# Autodesk Inventor assembly: Test_zebatek_odl_rowna_srednicy
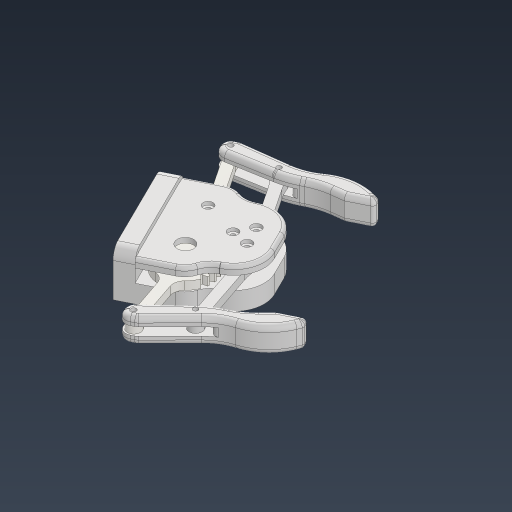
[picture p0: Inventor's stored thumbnail of the model, 512x512]
Saved by Autodesk Inventor 2024 (Build 280153000, 153)
## iProperties
Created: 2023-12-19
Part Number: Test_zebatek_odl_rowna_srednicy
Document SubType Name: Assembly
Designer: Piter
Author: Piter
## Documents named in this file (8)
- C:\Users\Piter\OneDrive\Pulpit\Modele\My-3D-printing-projects\gripper\Mygripper\Test_chwytaka.iam
- C:\Users\Piter\OneDrive\Pulpit\Modele\My-3D-printing-projects\gripper\Mygripper\Zebatka_servo.ipt
- C:\Users\Piter\OneDrive\Pulpit\Modele\My-3D-printing-projects\gripper\Mygripper\Podstawa.ipt
- C:\Users\Piter\OneDrive\Pulpit\Modele\My-3D-printing-projects\gripper\Mygripper\Connector.ipt
- C:\Users\Piter\OneDrive\Pulpit\Modele\My-3D-printing-projects\gripper\Mygripper\szczeka.ipt
- C:\Users\Piter\OneDrive\Pulpit\Modele\My-3D-printing-projects\gripper\Mygripper\Zebatka_bez_servo.ipt
- C:\Users\Piter\OneDrive\Pulpit\Modele\My-3D-printing-projects\gripper\Mygripper\Spacer.ipt
- C:\Users\Piter\OneDrive\Pulpit\Modele\My-3D-printing-projects\gripper\Mygripper\Top.ipt
## Components (9 placed, 6 different names)
1. Spur Gear2:2 — Rotational:1, Rotational:4, Mate:1, Mate:3, Rotational:5, Rotational:10, Rotation:1
2. Podstawa:1 — Rotational:1, Rotational:3, Rotational:4, Rotational:8, Rotational:9, Rotational:10, Rigid:1, Mate:7, Mate:8, Mate:9
3. Connector:1 — Rotational:3, Mate:2, Mate:4
4. Connector:2 — Rotational:8, Mate:5
5. szczeka:1 — Mate:1, Mate:2, Mate:3, Rotational:5, Mate:4
6. szczeka:2 — Mate:5, Mate:6
7. Spur Gear2:3 — Rotational:9, Mate:6, Rotation:1
8. Spacer:1 — Rigid:1
9. Top:1 — Mate:7, Mate:8, Mate:9
## Relationships (18: Mate 9, RevoluteJoint 7, RelateRotation 1, WeldJoint 1)
- Rotational:1 [RevoluteJoint]: Spur Gear2:2 ↔ Podstawa:1
- Rotational:3 [RevoluteJoint]: Podstawa:1 ↔ Connector:1
- Rotational:4 [RevoluteJoint]: Spur Gear2:2 ↔ Podstawa:1
- Mate:1: Spur Gear2:2 ↔ szczeka:1
- Mate:2: Connector:1 ↔ szczeka:1
- Mate:3: Spur Gear2:2 ↔ szczeka:1
- Rotational:5 [RevoluteJoint]: Spur Gear2:2 ↔ szczeka:1
- Mate:4: Connector:1 ↔ szczeka:1
- Rotational:8 [RevoluteJoint]: Podstawa:1 ↔ Connector:2
- Mate:5: Connector:2 ↔ szczeka:2
- Rotational:9 [RevoluteJoint]: Podstawa:1 ↔ Spur Gear2:3
- Mate:6: szczeka:2 ↔ Spur Gear2:3
- Rotational:10 [RevoluteJoint]: Spur Gear2:2 ↔ Podstawa:1
- Rotation:1 [RelateRotation] (1 ul): Spur Gear2:2 ↔ Spur Gear2:3
- Rigid:1 [WeldJoint]: Podstawa:1 ↔ Spacer:1
- Mate:7: Podstawa:1 ↔ Top:1
- Mate:8: Podstawa:1 ↔ Top:1
- Mate:9: Podstawa:1 ↔ Top:1
